# Autodesk Inventor assembly: Zespół1
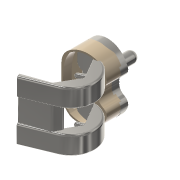
[picture p0: Inventor's stored thumbnail of the model, 180x180]
Saved by Autodesk Inventor 2017 (Build 210142000, 142)
## iProperties
Part Number: Zespół1
Material: Ogólny
Document SubType Name: Assembly
Designer: Kinga Nowak
Engr Approved By: dr Marta Kiel-Jamrozik
Description: Endoproteza stawu kolanowego
Mfg Approved By: dr Marta Kiel-Jarmozik
Authority: dr Marta Kiel-Jamrozik
Author: kinga
## Documents named in this file (4)
- C:\Users\kinga\Desktop\uczelnia\semestr VI\implanty\projekt\Zespół1.iam
- C:\Users\kinga\Desktop\uczelnia\semestr VI\implanty\projekt\czesc-piszczelowa.ipt
- C:\Users\kinga\Desktop\uczelnia\semestr VI\implanty\projekt\czesc-udowa.ipt
- C:\Users\kinga\Desktop\uczelnia\semestr VI\implanty\projekt\wkladka.ipt
## Components (3 placed, 3 different names)
1. czesc-piszczelowa:1 — Zestawiający:1, Równoległy:1
2. czesc-udowa:1 — Zestawiający:2
3. wkladka:1 — Zestawiający:1, Równoległy:1, Zestawiający:2
## Relationships (3: Mate 2, Flush 1)
- Zestawiający:1 [Mate]: czesc-piszczelowa:1 ↔ wkladka:1
- Równoległy:1 [Flush]: czesc-piszczelowa:1 ↔ wkladka:1
- Zestawiający:2 [Mate]: czesc-udowa:1 ↔ wkladka:1
